# Autodesk Inventor assembly: Assembly1
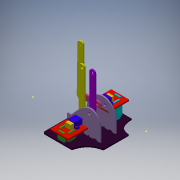
[picture p0: Inventor's stored thumbnail of the model, 180x180]
Saved by Autodesk Inventor 2016 (Build 200138000, 138)
## iProperties
Created: 2017-09-18
Part Number: Assembly1
Document SubType Name: Assembly
Designer: student
Author: student
## Documents named in this file (18)
- C:\Users\student\Documents\Inventor Files\arm4\Assembly1.iam
- C:\Users\student\Documents\Inventor Files\arm4\arm4_2.ipt
- C:\Users\student\Documents\Inventor Files\arm4\arm4_3.ipt
- C:\Users\student\Documents\Inventor Files\arm4\arm4_4.ipt
- C:\Users\student\Documents\Inventor Files\arm4\arm4_5.ipt
- C:\Users\student\Documents\Inventor Files\arm4\arm4_6.ipt
- C:\Users\student\Documents\Inventor Files\arm4\amr4_7.ipt
- C:\Users\student\Documents\Inventor Files\arm4\arm4_13.ipt
- C:\Users\student\Documents\Inventor Files\arm4\Part5.ipt
- C:\Users\student\Documents\Inventor Files\arm4\arm4_8.ipt
- C:\Users\student\Documents\Inventor Files\arm4\mini_motor.ipt
- C:\Users\student\Documents\Inventor Files\arm4\Part10.ipt
- C:\Users\student\Documents\Inventor Files\arm4\arm4_11.ipt
- C:\Users\student\Documents\Inventor Files\arm4\arm4_12.ipt
- C:\Users\student\Documents\Inventor Files\arm4\arpm4_14.ipt
- C:\Users\student\Documents\Inventor Files\arm4\Part2.ipt
- C:\Users\student\Documents\Inventor Files\arm4\Part3.ipt
- C:\Users\student\Documents\Inventor Files\arm4\Part4.ipt
## Components (46 placed, 17 different names)
1. arm4_3:1 — Rotational:1, Angle:2, Rigid:4, Rigid:8, Rigid:9, Rigid:10, Rigid:13, Rigid:17
2. arm4_2:1 — Rotational:1, Angle:1, Rigid:33, Rotational:11
3. arm4_2:2 — Rotational:3, Angle:3, Rigid:14, Rigid:15, Rigid:16, Rotational:6
4. arm4_4:1 — Rotational:4, Angle:4
5. arm4_6:1 — Rigid:4
6. arm4_6:3 — Rigid:6
7. arm4_6:4 — Rigid:8, Rotational:3
8. arm4_6:5 — Rigid:9, Rigid:31
9. arm4_6:6 — Rigid:10, Rotational:7
10. arm4_6:7 — Rigid:13
11. arm4_6:8 — Rigid:14
12. amr4_7:1 — Rotational:6, Rigid:22, Angle:5
13. arm4_6:9 — Rigid:15
14. arm4_5:4 — Rigid:16
15. arm4_5:5 — Rigid:17, Rigid:21, Rigid:30
16. arm4_6:10 — Rigid:21, Rigid:25
17. arm4_6:11 — Rigid:20, Rigid:22, Rigid:23, Rotational:8
18. arm4_6:12 — Rigid:23
19. arm4_5:6 — Rigid:20, Rigid:26
20. arm4_13:1 — Rotational:7, Rotational:8, Rigid:24, Rigid:27
21. arm4_2:3 — Rotational:9, Angle:6, Rotational:10
22. arm4_6:13 — Rigid:24, Rotational:9
23. arm4_5:7 — Rigid:25
24. arm4_5:8 — Rigid:26, Rigid:29
25. arm4_6:14 — Rigid:27, Rigid:28
26. arm4_5:9 — Rigid:28
27. arm4_5:10 — Rigid:30
28. arm4_5:11 — Rigid:29
29. arm4_5:12 — Rigid:31
30. Part5:1 — Rotational:10, Angle:7, Rotational:12
31. arm4_8:1 — Rigid:33, Flush:1
32. mini_motor:1 — Rotational:11, Angle:8, Mate:12, Mate:16, Angle:9, Angle:11
33. mini_motor:2 — Rotational:12, Mate:1, Mate:2, Mate:5, Rigid:37, Mate:21, Mate:22
34. Part10:1 — Mate:18, Angle:10, Mate:20, Angle:11
35. Part10:2 — Mate:1, Mate:2, Mate:5
36. arm4_12:1 — Flush:1, Mate:20, Rigid:6, Rotational:4, Flush:2
37. arm4_11:2 — Mate:12, Rigid:34, Rigid:35, Rigid:36
38. arpm4_14:2 — Rigid:34
39. arpm4_14:3 — Rigid:35
40. arpm4_14:4 — Rigid:36
41. Part2:1 — Angle:12, Angle:13, Rigid:37, Mate:23
42. arm4_11:3 — Mate:21, Mate:22, Mate:23, Rigid:38, Rigid:39, Rigid:40
43. Part3:1 — Rigid:38
44. Part3:2 — Rigid:40
45. Part3:3 — Rigid:39
46. Part4:1 — Flush:2
## Relationships (66: WeldJoint 30, Angle 13, Mate 11, RevoluteJoint 10, Flush 2)
- Rotational:1 [RevoluteJoint] (-0.762 mm): arm4_3:1 ↔ arm4_2:1
- Angle:1 (180 deg): arm4_2:1
- Angle:2 (0 deg): arm4_3:1
- Rotational:3 [RevoluteJoint] (0.762 mm): arm4_2:2 ↔ arm4_6:4
- Angle:3 (180 deg): arm4_2:2
- Rotational:4 [RevoluteJoint] (-3.937 mm): arm4_4:1 ↔ arm4_12:1
- Angle:4 (0 deg): arm4_4:1
- Rigid:4 [WeldJoint]: arm4_3:1 ↔ arm4_6:1
- Rigid:6 [WeldJoint]: arm4_6:3 ↔ arm4_12:1
- Rigid:8 [WeldJoint]: arm4_3:1 ↔ arm4_6:4
- Rigid:9 [WeldJoint]: arm4_3:1 ↔ arm4_6:5
- Rigid:10 [WeldJoint]: arm4_3:1 ↔ arm4_6:6
- Rigid:13 [WeldJoint] (-3.937 mm): arm4_3:1 ↔ arm4_6:7
- Rigid:14 [WeldJoint]: arm4_2:2 ↔ arm4_6:8
- Rigid:15 [WeldJoint] (-3.937 mm): arm4_2:2 ↔ arm4_6:9
- Rigid:16 [WeldJoint] (-4.699 mm): arm4_2:2 ↔ arm4_5:4
- Rigid:17 [WeldJoint] (-0.762 mm): arm4_3:1 ↔ arm4_5:5
- Rigid:20 [WeldJoint] (0.762 mm): arm4_6:11 ↔ arm4_5:6
- Rigid:21 [WeldJoint] (-6.35 mm): arm4_5:5 ↔ arm4_6:10
- Rotational:6 [RevoluteJoint] (-0.762 mm): arm4_2:2 ↔ amr4_7:1
- Rigid:22 [WeldJoint]: amr4_7:1 ↔ arm4_6:11
- Rigid:23 [WeldJoint] (10.287 mm): arm4_6:11 ↔ arm4_6:12
- Angle:5 (180 deg): amr4_7:1
- Rotational:7 [RevoluteJoint] (11.049 mm): arm4_6:6 ↔ arm4_13:1
- Rotational:8 [RevoluteJoint] (11.049 mm): arm4_6:11 ↔ arm4_13:1
- Rigid:24 [WeldJoint]: arm4_13:1 ↔ arm4_6:13
- Rotational:9 [RevoluteJoint] (0.762 mm): arm4_2:3 ↔ arm4_6:13
- Angle:6 (0 deg): arm4_2:3
- Rigid:25 [WeldJoint]: arm4_6:10 ↔ arm4_5:7
- Rigid:26 [WeldJoint]: arm4_5:6 ↔ arm4_5:8
- Rigid:27 [WeldJoint]: arm4_13:1 ↔ arm4_6:14
- Rigid:28 [WeldJoint] (0.762 mm): arm4_6:14 ↔ arm4_5:9
- Rigid:29 [WeldJoint]: arm4_5:8 ↔ arm4_5:11
- Rigid:30 [WeldJoint]: arm4_5:5 ↔ arm4_5:10
- Rigid:31 [WeldJoint]: arm4_6:5 ↔ arm4_5:12
- Rotational:10 [RevoluteJoint]: arm4_2:3 ↔ Part5:1
- Angle:7 (0 deg): Part5:1
- Rigid:33 [WeldJoint] (3.175 mm): arm4_2:1 ↔ arm4_8:1
- Rotational:11 [RevoluteJoint] (-0.635 mm): arm4_2:1 ↔ mini_motor:1
- Rotational:12 [RevoluteJoint] (-3.81 mm): Part5:1 ↔ mini_motor:2
- Angle:8 (0 deg): mini_motor:1
- Mate:1: mini_motor:2 ↔ Part10:2
- Mate:2: mini_motor:2 ↔ Part10:2
- Mate:5: mini_motor:2 ↔ Part10:2
- Flush:1: arm4_8:1 ↔ arm4_12:1
- Mate:12: mini_motor:1 ↔ arm4_11:2
- Mate:16: mini_motor:1
- Angle:9 (0 deg): mini_motor:1
- Mate:18: Part10:1
- Angle:10 (0 deg): Part10:1
- Mate:19
- Mate:20: Part10:1 ↔ arm4_12:1
- Angle:11 (180 deg): mini_motor:1 ↔ Part10:1
- Rigid:34 [WeldJoint] (1.397 mm): arm4_11:2 ↔ arpm4_14:2
- Rigid:35 [WeldJoint] (1.397 mm): arm4_11:2 ↔ arpm4_14:3
- Rigid:36 [WeldJoint] (1.397 mm): arm4_11:2 ↔ arpm4_14:4
- Angle:12 (180 deg): Part2:1
- Angle:13 (0 deg): Part2:1
- Rigid:37 [WeldJoint]: mini_motor:2 ↔ Part2:1
- Mate:21: mini_motor:2 ↔ arm4_11:3
- Mate:22: mini_motor:2 ↔ arm4_11:3
- Mate:23 (-2.921 mm): Part2:1 ↔ arm4_11:3
- Rigid:38 [WeldJoint] (1.4027 mm): arm4_11:3 ↔ Part3:1
- Rigid:39 [WeldJoint]: arm4_11:3 ↔ Part3:3
- Rigid:40 [WeldJoint]: arm4_11:3 ↔ Part3:2
- Flush:2: arm4_12:1 ↔ Part4:1
